# Autodesk Inventor assembly: 組合4-16
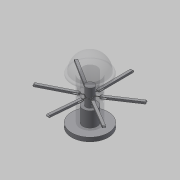
[picture p0: Inventor's stored thumbnail of the model, 180x180]
Saved by Autodesk Inventor 2018 (Build 220112000, 112)
## iProperties
Created: 2021-04-16
Part Number: 組合4-16
Material: 一般
Document SubType Name: Assembly
Designer: 王鼎鈞
Author: 王鼎鈞
## Documents named in this file (4)
- D:\2021顏家民\四人圖檔\組合4-16.iam
- D:\2021顏家民\四人圖檔\3d凸輪4-16.ipt
- D:\2021顏家民\四人圖檔\支架4-16.ipt
- D:\2021顏家民\四人圖檔\主體4-15.ipt
## Components (8 placed, 3 different names)
1. 3d凸輪4-16:1 — 插入:1, 相切:1, 相切:3, 旋轉:1, 相切:8, 相切:9, 相切:18, 相切:19, 相切:20, 相切:21, 相切:22, 相切:23, 相切:24, 相切:25
2. 支架4-16:1 — 相切:1, 貼合:1, 相切:3, 相切:4, 相切:5
3. 主體4-15:1 — 插入:1, 貼合:1, 相切:4, 旋轉:1, 相切:5, 貼合:2, 相切:6, 相切:7, 貼合:3, 相切:10, 相切:11, 貼合:4, 相切:12, 相切:13, 貼合:5, 相切:14, 相切:15, 貼合:6, 相切:16, 相切:17
4. 支架4-16:2 — 貼合:2, 相切:6, 相切:7, 相切:8, 相切:9
5. 支架4-16:3 — 貼合:3, 相切:10, 相切:11, 相切:18, 相切:19
6. 支架4-16:4 — 貼合:4, 相切:12, 相切:13, 相切:20, 相切:21
7. 支架4-16:6 — 貼合:6, 相切:16, 相切:17, 相切:24, 相切:25
8. 支架4-16:7 — 貼合:5, 相切:14, 相切:15, 相切:22, 相切:23
## Relationships (32: Tangent 24, Mate 6, Insert 1, RevoluteJoint 1)
- 插入:1 [Insert]: 3d凸輪4-16:1 ↔ 主體4-15:1
- 相切:1 [Tangent]: 3d凸輪4-16:1 ↔ 支架4-16:1
- 貼合:1 [Mate]: 支架4-16:1 ↔ 主體4-15:1
- 相切:3 [Tangent]: 3d凸輪4-16:1 ↔ 支架4-16:1
- 相切:4 [Tangent]: 支架4-16:1 ↔ 主體4-15:1
- 旋轉:1 [RevoluteJoint]: 3d凸輪4-16:1 ↔ 主體4-15:1
- 相切:5 [Tangent]: 支架4-16:1 ↔ 主體4-15:1
- 貼合:2 [Mate]: 主體4-15:1 ↔ 支架4-16:2
- 相切:6 [Tangent]: 主體4-15:1 ↔ 支架4-16:2
- 相切:7 [Tangent]: 主體4-15:1 ↔ 支架4-16:2
- 相切:8 [Tangent]: 3d凸輪4-16:1 ↔ 支架4-16:2
- 相切:9 [Tangent]: 3d凸輪4-16:1 ↔ 支架4-16:2
- 貼合:3 [Mate]: 主體4-15:1 ↔ 支架4-16:3
- 相切:10 [Tangent]: 主體4-15:1 ↔ 支架4-16:3
- 相切:11 [Tangent]: 主體4-15:1 ↔ 支架4-16:3
- 貼合:4 [Mate]: 主體4-15:1 ↔ 支架4-16:4
- 相切:12 [Tangent]: 主體4-15:1 ↔ 支架4-16:4
- 相切:13 [Tangent]: 主體4-15:1 ↔ 支架4-16:4
- 貼合:5 [Mate]: 主體4-15:1 ↔ 支架4-16:7
- 相切:14 [Tangent]: 主體4-15:1 ↔ 支架4-16:7
- 相切:15 [Tangent]: 主體4-15:1 ↔ 支架4-16:7
- 貼合:6 [Mate]: 主體4-15:1 ↔ 支架4-16:6
- 相切:16 [Tangent]: 主體4-15:1 ↔ 支架4-16:6
- 相切:17 [Tangent]: 主體4-15:1 ↔ 支架4-16:6
- 相切:18 [Tangent]: 3d凸輪4-16:1 ↔ 支架4-16:3
- 相切:19 [Tangent]: 3d凸輪4-16:1 ↔ 支架4-16:3
- 相切:20 [Tangent]: 3d凸輪4-16:1 ↔ 支架4-16:4
- 相切:21 [Tangent]: 3d凸輪4-16:1 ↔ 支架4-16:4
- 相切:22 [Tangent]: 3d凸輪4-16:1 ↔ 支架4-16:7
- 相切:23 [Tangent]: 3d凸輪4-16:1 ↔ 支架4-16:7
- 相切:24 [Tangent]: 3d凸輪4-16:1 ↔ 支架4-16:6
- 相切:25 [Tangent]: 3d凸輪4-16:1 ↔ 支架4-16:6
